# Autodesk Inventor assembly: wheel2
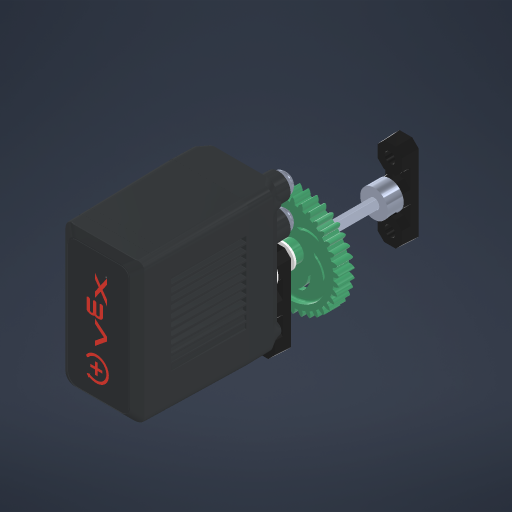
[picture p0: Inventor's stored thumbnail of the model, 512x512]
Saved by Autodesk Inventor 2024 (Build 280153000, 153)
## iProperties
Created: 2023-08-09
Part Number: wheel2
Document SubType Name: Assembly
Designer: macbook
Author: macbook
## Documents named in this file (13)
- \\Mac\Home\Desktop\code\7899V-VRC-OVER-UNDER\Cad\VEX-CAD-Inventor-1.4.0\Assembly\v0.2\wheel2.iam
- \\Mac\Home\Desktop\code\7899V-VRC-OVER-UNDER\Cad\VEX-CAD-Inventor-1.4.0\Motion\Gears\LS 36T Gear.ipt
- \\Mac\Home\Desktop\code\7899V-VRC-OVER-UNDER\Cad\VEX-CAD-Inventor-1.4.0\Motion\Shaft LS\Bearing Flat.ipt
- \\Mac\Home\Desktop\code\7899V-VRC-OVER-UNDER\Cad\VEX-CAD-Inventor-1.4.0\Motion\Shaft LS\Shaft LS.ipt
- \\Mac\Home\Desktop\code\7899V-VRC-OVER-UNDER\Cad\VEX-CAD-Inventor-1.4.0\Motion\Shaft LS\Shaft Collar Metal.iam
- \\Mac\Home\Desktop\code\7899V-VRC-OVER-UNDER\Cad\VEX-CAD-Inventor-1.4.0\Electronics\Motors with Screws\AluM-StarS.iam
- \\Mac\Home\Desktop\code\7899V-VRC-OVER-UNDER\Cad\VEX-CAD-Inventor-1.4.0\Electronics\Motors with Screws.iam
- \\Mac\Home\Desktop\code\7899V-VRC-OVER-UNDER\Cad\VEX-CAD-Inventor-1.4.0\Motion\Spacers\Spacer Nylon .500 OD.ipt
- \\Mac\Home\Desktop\code\7899V-VRC-OVER-UNDER\Cad\VEX-CAD-Inventor-1.4.0\Motion\Shaft LS\Shaft Collar Metal\Shaft Collar Set Screw.iam
- \\Mac\Home\Desktop\code\7899V-VRC-OVER-UNDER\Cad\VEX-CAD-Inventor-1.4.0\Motion\Spacers\Spacer Nylon .500 OD\NSpacer White .500 OD x .125.ipt
- \\Mac\Home\Desktop\code\7899V-VRC-OVER-UNDER\Cad\VEX-CAD-Inventor-1.4.0\Motion\Shaft LS\Shaft LS\Shaft LS 3.0.ipt
- \\Mac\Home\Desktop\code\7899V-VRC-OVER-UNDER\Cad\VEX-CAD-Inventor-1.4.0\Motion\Spacers\Washer Teflon\TWasher .375 OD x .03125.ipt
- \\Mac\Home\Desktop\code\7899V-VRC-OVER-UNDER\Cad\VEX-CAD-Inventor-1.4.0\Motion\Spacers\Washer Teflon.ipt
## Components (9 placed, 7 different names)
1. LS 36T Gear:1
2. Shaft LS 3.0:1 — Cylindrical:2, Mate:1
3. Shaft Collar Set Screw:1 [sub-assembly] — Insert:22
4. Shaft Collar Set Screw:2 [sub-assembly] — Cylindrical:2
5. AluM-StarS:1 [sub-assembly] — Mate:1, Insert:20, Flush:1
6. TWasher .375 OD x .03125:1
7. Bearing Flat:3 — Insert:19, Flush:1, Insert:21
8. NSpacer White .500 OD x .125:1 — Insert:19
9. Bearing Flat:4 — Insert:20, Insert:21, Insert:22
## Relationships (10: Insert 7, CylindricalJoint 1, Mate 1, Flush 1)
- [Insert]: LS 36T Gear:1 ↔ TWasher .375 OD x .03125:1
- [Insert]: LS 36T Gear:1 ↔ Shaft Collar Set Screw:2
- Cylindrical:2: Shaft LS 3.0:1 ↔ Shaft Collar Set Screw:2
- Mate:1: Shaft LS 3.0:1 ↔ AluM-StarS:1
- [Insert] (1.5875 mm): TWasher .375 OD x .03125:1 ↔ Bearing Flat:3
- Insert:19: Bearing Flat:3 ↔ NSpacer White .500 OD x .125:1
- Insert:20 (42.8625 mm): AluM-StarS:1 ↔ Bearing Flat:4
- Flush:1: AluM-StarS:1 ↔ Bearing Flat:3
- Insert:21 (44.45 mm): Bearing Flat:3 ↔ Bearing Flat:4
- Insert:22: Shaft Collar Set Screw:1 ↔ Bearing Flat:4
